# Autodesk Inventor assembly: Assembly
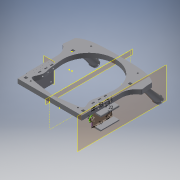
[picture p0: Inventor's stored thumbnail of the model, 180x180]
Saved by Autodesk Inventor 2019 (Build 230136000, 136)
## iProperties
Created: 2019-04-08
Part Number: Assembly
Material: Ogólny
Document SubType Name: Assembly
Designer: terg
Author: terg
## Documents named in this file (5)
- D:\Projekt\Projekt---platforma-mobilna\Chassis\Assembly.iam
- D:\Projekt\Projekt---platforma-mobilna\Chassis\base.ipt
- D:\Projekt\Projekt---platforma-mobilna\Chassis\motor_grip_L.ipt
- D:\Projekt\Projekt---platforma-mobilna\Chassis\motor_grip_R.ipt
- D:\Projekt\Projekt---platforma-mobilna\Chassis\wheel.ipt
## Components (5 placed, 4 different names)
1. base:1 — Płaskie:1, Płaskie:2, Obrotowe:1, Obrotowe:2, Zestawiający:1, Zestawiający:2
2. motor_grip_L:1 — Płaskie:1
3. motor_grip_R:1 — Płaskie:2
4. wheel:1 — Obrotowe:2, Zestawiający:1
5. wheel:2 — Obrotowe:1, Zestawiający:2
## Relationships (6: PlanarJoint 2, RevoluteJoint 2, Mate 2)
- Płaskie:1 [PlanarJoint]: base:1 ↔ motor_grip_L:1
- Płaskie:2 [PlanarJoint]: base:1 ↔ motor_grip_R:1
- Obrotowe:1 [RevoluteJoint] (1 mm): base:1 ↔ wheel:2
- Obrotowe:2 [RevoluteJoint] (-1 mm): base:1 ↔ wheel:1
- Zestawiający:1 [Mate]: base:1 ↔ wheel:1
- Zestawiający:2 [Mate]: base:1 ↔ wheel:2
